# Autodesk Inventor assembly: fight_robot
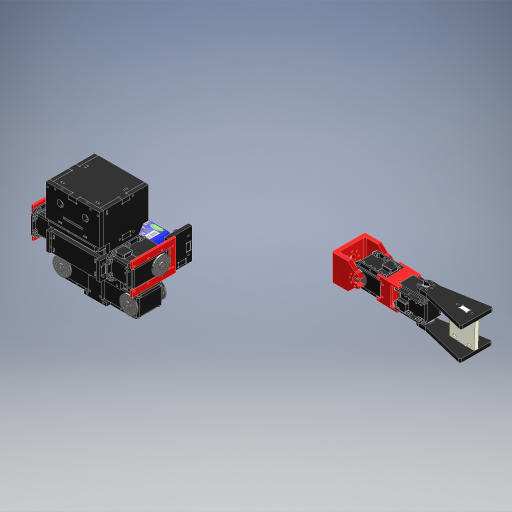
[picture p0: Inventor's stored thumbnail of the model, 512x512]
Saved by Autodesk Inventor 2024 (Build 280153000, 153)
## iProperties
Created: 2024-09-15
Part Number: fight_robot
Document SubType Name: Assembly
Designer: msi
Author: msi
## Documents named in this file (4)
- C:\Users\msi\GITHUB\19th_intern_kgh_fight_robot\부품\fight_robot.iam
- C:\Users\msi\GITHUB\19th_intern_kgh_fight_robot\부품\Upper_body\Body\body.iam
- C:\Users\msi\GITHUB\19th_intern_kgh_fight_robot\부품\Upper_body\Arm\arm_left.iam
- C:\Users\msi\GITHUB\19th_intern_kgh_fight_robot\부품\Lower_Body\Hip_joint\hip_joint.iam
## Components (3 placed, 3 different names)
1. arm_left:1 [sub-assembly]
2. hip_joint:1 [sub-assembly] — 삽입:1, 삽입:2
3. body:1 [sub-assembly] — 삽입:1, 삽입:2
## Relationships (2: Insert 2)
- 삽입:1 [Insert]: hip_joint:1 ↔ body:1
- 삽입:2 [Insert]: hip_joint:1 ↔ body:1
